# Autodesk Inventor assembly: HbthumbU01
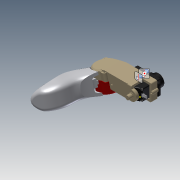
[picture p0: Inventor's stored thumbnail of the model, 180x180]
Saved by Autodesk Inventor 2015 SP1 (Build 190203100, 203)
## iProperties
Created: 2015-02-19
Part Number: HbthumbU01
Document SubType Name: Assembly
Designer: Yamaura
Author: Yamaura
## Documents named in this file (9)
- C:\Users\Yamaura\Documents\GitHub\HACKberry\HACKberry-hardware\3D\Inventor\Parts\HbthumbU01.iam
- C:\Users\Yamaura\Documents\GitHub\HACKberry\HACKberry-hardware\3D\Inventor\Parts\ASV-15MG.ipt
- C:\Users\Yamaura\Documents\GitHub\HACKberry\HACKberry-hardware\3D\Inventor\Parts\ScrewM2L8.ipt
- C:\Users\Yamaura\Documents\GitHub\HACKberry\HACKberry-hardware\3D\Inventor\Parts\Hbthumb04.ipt
- C:\Users\Yamaura\Documents\GitHub\HACKberry\HACKberry-hardware\3D\Inventor\Parts\HbThumbLockButton01.ipt
- C:\Users\Yamaura\Documents\GitHub\HACKberry\HACKberry-hardware\3D\Inventor\Parts\HbThumbProximalPhalanx01.ipt
- C:\Users\Yamaura\Documents\GitHub\HACKberry\HACKberry-hardware\3D\Inventor\Parts\HbThumbMetacarpalPhalanx01.ipt
- C:\Users\Yamaura\Documents\GitHub\HACKberry\HACKberry-hardware\3D\Inventor\Parts\HbThumbMetacarpalPhalanxCover01.ipt
- C:\Users\Yamaura\Documents\GitHub\HACKberry\HACKberry-hardware\3D\Inventor\Parts\CP 0.5-6-8.ipt
## Components (9 placed, 8 different names)
1. ASV-15MG:1 — フラッシュ:1, メイト:1, 角度:1, メイト:4, メイト:5, メイト:6, メイト:7, メイト:16, メイト:17, メイト:18
2. ScrewM2L8:1 — メイト:4, メイト:5
3. ScrewM2L8:2 — メイト:6, メイト:7
4. Hbthumb04:1 — フラッシュ:2, メイト:9, メイト:10, メイト:11, メイト:13, メイト:14, フラッシュ:17, メイト:16, メイト:17, メイト:18, 角度:3
5. HbThumbLockButton01:1 — メイト:12, メイト:13
6. HbThumbProximalPhalanx01:1 — メイト:11, フラッシュ:17, 角度:3
7. HbThumbMetacarpalPhalanx01:1 — フラッシュ:3, メイト:10, メイト:12, メイト:15, 角度:2
8. HbThumbMetacarpalPhalanxCover01:1 — メイト:8, メイト:9
9. CP 0.5-6-8:1 — メイト:14, メイト:15
## Relationships (23: Mate 16, Flush 4, Angle 3)
- フラッシュ:1 [Flush]: ASV-15MG:1
- メイト:1 [Mate]: ASV-15MG:1
- 角度:1 [Angle] (0 deg): ASV-15MG:1
- メイト:4 [Mate]: ASV-15MG:1 ↔ ScrewM2L8:1
- メイト:5 [Mate]: ASV-15MG:1 ↔ ScrewM2L8:1
- メイト:6 [Mate]: ASV-15MG:1 ↔ ScrewM2L8:2
- メイト:7 [Mate]: ASV-15MG:1 ↔ ScrewM2L8:2
- フラッシュ:2 [Flush] (8 mm): Hbthumb04:1
- メイト:8 [Mate]: HbThumbMetacarpalPhalanxCover01:1
- メイト:9 [Mate]: Hbthumb04:1 ↔ HbThumbMetacarpalPhalanxCover01:1
- フラッシュ:3 [Flush]: HbThumbMetacarpalPhalanx01:1
- メイト:10 [Mate]: Hbthumb04:1 ↔ HbThumbMetacarpalPhalanx01:1
- メイト:11 [Mate]: Hbthumb04:1 ↔ HbThumbProximalPhalanx01:1
- メイト:12 [Mate]: HbThumbLockButton01:1 ↔ HbThumbMetacarpalPhalanx01:1
- メイト:13 [Mate]: Hbthumb04:1 ↔ HbThumbLockButton01:1
- メイト:14 [Mate]: Hbthumb04:1 ↔ CP 0.5-6-8:1
- メイト:15 [Mate]: HbThumbMetacarpalPhalanx01:1 ↔ CP 0.5-6-8:1
- フラッシュ:17 [Flush]: Hbthumb04:1 ↔ HbThumbProximalPhalanx01:1
- メイト:16 [Mate]: ASV-15MG:1 ↔ Hbthumb04:1
- メイト:17 [Mate]: ASV-15MG:1 ↔ Hbthumb04:1
- メイト:18 [Mate]: ASV-15MG:1 ↔ Hbthumb04:1
- 角度:2 [Angle] (180 deg): HbThumbMetacarpalPhalanx01:1
- 角度:3 [Angle] (65 deg): Hbthumb04:1 ↔ HbThumbProximalPhalanx01:1
